# Autodesk Inventor assembly: 012896
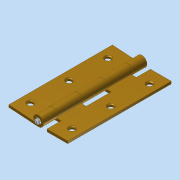
[picture p0: Inventor's stored thumbnail of the model, 180x180]
Saved by Autodesk Inventor 2012 SP1 (Build 160190100, 190)
## iProperties
Created: 2014-07-02
Part Number: 012896
Document SubType Name: Assembly
Designer: Eisele
Description: Schanier
Benennung: Schanier
Abmaße: 30x26x0,9
Author: Eisele
Title: 012896 Schanier
## Documents named in this file (3)
- C:\Users\eisele\Documents\Inventor privat\Projekte\Klapptisch\012896_Scharnier.iam
- C:\Users\eisele\Documents\Inventor privat\Projekte\Klapptisch\012894_a.ipt
- C:\Users\eisele\Documents\Inventor privat\Projekte\Klapptisch\012895_b.ipt
## Components (2 placed, 2 different names)
1. DIV / Schanier / 012894.ipt / Schanier A-Seite-012894:1 — Passend:1, Passend:2, Passend:4, Passend:5, Winkel:1, Winkel:2, Winkel:3
2. DIV / Schanier / 012895.ipt / Schanier B-Seite-012895:1 — Passend:2, Fluchtend:3, Winkel:1, Winkel:2, Winkel:3
## Relationships (8: Mate 4, Angle 3, Flush 1)
- Passend:1 [Mate]: DIV / Schanier / 012894.ipt / Schanier A-Seite-012894:1
- Passend:2 [Mate]: DIV / Schanier / 012894.ipt / Schanier A-Seite-012894:1 ↔ DIV / Schanier / 012895.ipt / Schanier B-Seite-012895:1
- Fluchtend:3 [Flush]: DIV / Schanier / 012895.ipt / Schanier B-Seite-012895:1
- Passend:4 [Mate]: DIV / Schanier / 012894.ipt / Schanier A-Seite-012894:1
- Passend:5 [Mate]: DIV / Schanier / 012894.ipt / Schanier A-Seite-012894:1
- Winkel:1 [Angle] (192 deg): DIV / Schanier / 012894.ipt / Schanier A-Seite-012894:1 ↔ DIV / Schanier / 012895.ipt / Schanier B-Seite-012895:1
- Winkel:2 [Angle] (105 deg): DIV / Schanier / 012894.ipt / Schanier A-Seite-012894:1 ↔ DIV / Schanier / 012895.ipt / Schanier B-Seite-012895:1
- Winkel:3 [Angle] (0 deg): DIV / Schanier / 012894.ipt / Schanier A-Seite-012894:1 ↔ DIV / Schanier / 012895.ipt / Schanier B-Seite-012895:1
